# Autodesk Inventor assembly: fc16-080
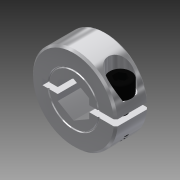
[picture p0: Inventor's stored thumbnail of the model, 180x180]
Saved by Autodesk Inventor 2016 SP1 (Build 200210100, 210)
## iProperties
Category: Shaft Collars
Company: Autodesk Inc.
Created: 2015-12-04
Part Number: fc16-080
Document SubType Name: Assembly
Designer: Autodesk Inc.
Catalog Web Link: http://www.ruland.com/shaft-collar.php?recordID=CL-6HX-A
Vendor: Ruland
Author: Autodesk Inc.
Keywords: FIRSTChoice
## Documents named in this file (3)
- D:\FIRST\FRC KOP 2016\FRC FIRSTChoice 2016\fc16-080_ShaftCollar.iam
- D:\FIRST\FRC KOP 2016\FRC FIRSTChoice 2016\Parts\MISC_ShaftCollar_CL-6HX-A.ipt
- D:\FIRST\FRC KOP 2016\FRC FIRSTChoice 2016\Parts\ANSI B18.3 - 6-32 UNC - 0.375(31).ipt
## Components (2 placed, 2 different names)
1. MISC_ShaftCollar_CL-6HX-A:1 — Insert:1
2. Hexagon Socket Head Cap Screw - Inch No. 6 - 32 UNC - 3/8:1 — Insert:1
## Relationships (1: Insert 1)
- Insert:1: MISC_ShaftCollar_CL-6HX-A:1 ↔ Hexagon Socket Head Cap Screw - Inch No. 6 - 32 UNC - 3/8:1
